# Autodesk Inventor assembly: STAGE1,ELEVATOR
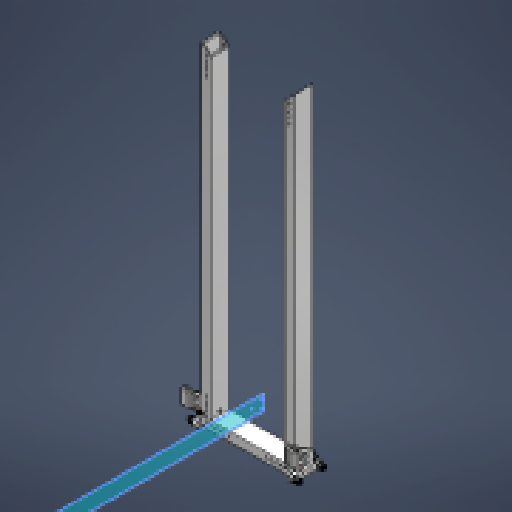
[picture p0: Inventor's stored thumbnail of the model, 512x512]
Saved by Autodesk Inventor 2024.3 (Build 283343000, 343)
## iProperties
ILogicPurgeVersion: 0.0.0.0
OnSaveVersion: 3.5.0.0
OnSaveAssembly: COREAutomationManager
Created: 2025-02-04
Part Number: STAGE1,ELEVATOR
Document SubType Name: Assembly
Designer: Jthib
Mfg Approved By: John.Thibert
Mass: 3994.13 g
Surface Area: 7109.04 cm^2
Volume: 1189.37 cm^3
Density: 3.3582 g/cm^3
ModelCat: Uncategorized
CN_MASS: 3.99
Author: Jthib
## Documents named in this file (12)
- \\clfs\homes\john.thibert\2025-Poseidon-Mechanical\STAGE1,ELEVATOR.iam
- \\clfs\homes\john.thibert\2025-Poseidon-Mechanical\TUBE,ELEVATOR,SIDE,STAGE1.ipt
- \\clfs\homes\john.thibert\2025-Poseidon-Mechanical\TUBE,ELEVATOR,BOT,STAGE1.ipt
- \\clfs\homes\john.thibert\2025-Poseidon-Mechanical\PLATE,BRACKET,ELEVATOR,STAGE1.ipt
- \\clfs\homes\john.thibert\2025-Poseidon-Mechanical\SLIDE,ELEVATOR,STAGE1,LH.iam
- \\clfs\homes\john.thibert\2025-Poseidon-Mechanical\SLIDE,ELEVATOR,STAGE1,RH.iam
- \\clfs\homes\john.thibert\2025-Poseidon-Mechanical\BRACE,CHAIN,#25,ELEVATOR.ipt
- \\clfs\homes\john.thibert\2025-Poseidon-Mechanical\BLOCK,BEARING,ARM,ELEVATOR.ipt
- \\clfs\homes\john.thibert\2025-Poseidon-Mechanical\60355K336_Ball Bearing.ipt
- \\clfs\homes\john.thibert\2025-Poseidon-Mechanical\91259A171_Alloy Steel Shoulder Screw.ipt
- \\clfs\homes\john.thibert\2025-Poseidon-Mechanical\BEARING,MOUNT,SIDE,ELEVATOR,MIRR.ipt
- \\clfs\homes\john.thibert\2025-Poseidon-Mechanical\BEARING,MOUNT,SIDE,ELEVATOR.ipt
## Components (19 placed, 13 different names)
1. SLIDE,ELEVATOR,STAGE1,LH.iam:1 [sub-assembly] — Mate:15, Mate:16, Mate:17, Mate:18
2. SLIDE,ELEVATOR,STAGE1,RH.iam:1 [sub-assembly]
3. TUBE,ELEVATOR,BOT,STAGE1.ipt:1 — Mate:14, Mate:19, Mate:20, Mate:22, Mate:23
4. TUBE,ELEVATOR,SIDE,STAGE1.ipt:1 — Mate:13, Mate:21, Mate:28, Mate:29, Mate:30
5. TUBE,ELEVATOR,SIDE,STAGE1.ipt:2 — Mate:24, Mate:25, Mate:26, Mate:27
6. BRACE,CHAIN,#25,ELEVATOR.ipt:1
7. PLATE,BRACKET,ELEVATOR,STAGE1.ipt:2
8. PLATE,BRACKET,ELEVATOR,STAGE1.ipt:1
9. BRACE,CHAIN,#25,ELEVATOR:2 — Mate:16, Mate:17, Mate:18
10. PLATE,BRACKET,ELEVATOR,STAGE1:4 — Mate:19, Mate:20, Mate:21
11. PLATE,BRACKET,ELEVATOR,STAGE1:5 — Mate:22, Mate:23, Mate:24
12. BLOCK,BEARING,ARM,ELEVATOR:1 — Mate:25, Mate:26, Mate:27
13. BEARING,MOUNT,SIDE,ELEVATOR:1
14. 91259A171_Alloy Steel Shoulder Screw:2
15. 60355K336_Ball Bearing:2
16. BEARING,MOUNT,SIDE,ELEVATOR,MIRR:1
17. 60355K336_Ball Bearing:1
18. 91259A171_Alloy Steel Shoulder Screw:1
19. BLOCK,BEARING,ARM,ELEVATOR:2 — Mate:28, Mate:29, Mate:30
## Relationships (47: Mate 37, Insert 10)
- [Insert]: TUBE,ELEVATOR,BOT,STAGE1.ipt:1 ↔ PLATE,BRACKET,ELEVATOR,STAGE1.ipt:1
- [Insert]: TUBE,ELEVATOR,BOT,STAGE1.ipt:1 ↔ PLATE,BRACKET,ELEVATOR,STAGE1.ipt:1
- [Insert]: TUBE,ELEVATOR,BOT,STAGE1.ipt:1 ↔ PLATE,BRACKET,ELEVATOR,STAGE1.ipt:2
- [Insert]: TUBE,ELEVATOR,BOT,STAGE1.ipt:1 ↔ PLATE,BRACKET,ELEVATOR,STAGE1.ipt:2
- [Insert]: TUBE,ELEVATOR,SIDE,STAGE1.ipt:2 ↔ PLATE,BRACKET,ELEVATOR,STAGE1.ipt:2
- [Insert]: TUBE,ELEVATOR,SIDE,STAGE1.ipt:2 ↔ PLATE,BRACKET,ELEVATOR,STAGE1.ipt:2
- [Insert]: TUBE,ELEVATOR,SIDE,STAGE1.ipt:1 ↔ PLATE,BRACKET,ELEVATOR,STAGE1.ipt:1
- [Insert]: TUBE,ELEVATOR,SIDE,STAGE1.ipt:1 ↔ PLATE,BRACKET,ELEVATOR,STAGE1.ipt:1
- [Mate]: SLIDE,ELEVATOR,STAGE1,RH.iam:1 ↔ TUBE,ELEVATOR,SIDE,STAGE1.ipt:2
- [Mate]: SLIDE,ELEVATOR,STAGE1,RH.iam:1 ↔ TUBE,ELEVATOR,SIDE,STAGE1.ipt:2
- [Mate]: SLIDE,ELEVATOR,STAGE1,RH.iam:1 ↔ TUBE,ELEVATOR,SIDE,STAGE1.ipt:2
- [Mate]: SLIDE,ELEVATOR,STAGE1,LH.iam:1 ↔ TUBE,ELEVATOR,SIDE,STAGE1.ipt:1
- [Mate]: SLIDE,ELEVATOR,STAGE1,LH.iam:1 ↔ TUBE,ELEVATOR,SIDE,STAGE1.ipt:1
- [Mate]: SLIDE,ELEVATOR,STAGE1,LH.iam:1 ↔ TUBE,ELEVATOR,SIDE,STAGE1.ipt:1
- [Mate]: SLIDE,ELEVATOR,STAGE1,RH.iam:1 ↔ BRACE,CHAIN,#25,ELEVATOR.ipt:1
- [Mate]: SLIDE,ELEVATOR,STAGE1,RH.iam:1 ↔ BRACE,CHAIN,#25,ELEVATOR.ipt:1
- [Mate]: SLIDE,ELEVATOR,STAGE1,RH.iam:1 ↔ BRACE,CHAIN,#25,ELEVATOR.ipt:1
- Mate:13 (-127 mm): TUBE,ELEVATOR,SIDE,STAGE1.ipt:1
- Mate:14 (-457.2 mm): TUBE,ELEVATOR,BOT,STAGE1.ipt:1
- Mate:15: SLIDE,ELEVATOR,STAGE1,LH.iam:1
- Mate:16: SLIDE,ELEVATOR,STAGE1,LH.iam:1 ↔ BRACE,CHAIN,#25,ELEVATOR:2
- Mate:17: SLIDE,ELEVATOR,STAGE1,LH.iam:1 ↔ BRACE,CHAIN,#25,ELEVATOR:2
- Mate:18: SLIDE,ELEVATOR,STAGE1,LH.iam:1 ↔ BRACE,CHAIN,#25,ELEVATOR:2
- Mate:19: TUBE,ELEVATOR,BOT,STAGE1.ipt:1 ↔ PLATE,BRACKET,ELEVATOR,STAGE1:4
- Mate:20: TUBE,ELEVATOR,BOT,STAGE1.ipt:1 ↔ PLATE,BRACKET,ELEVATOR,STAGE1:4
- Mate:21: TUBE,ELEVATOR,SIDE,STAGE1.ipt:1 ↔ PLATE,BRACKET,ELEVATOR,STAGE1:4
- Mate:22: TUBE,ELEVATOR,BOT,STAGE1.ipt:1 ↔ PLATE,BRACKET,ELEVATOR,STAGE1:5
- Mate:23: TUBE,ELEVATOR,BOT,STAGE1.ipt:1 ↔ PLATE,BRACKET,ELEVATOR,STAGE1:5
- Mate:24: TUBE,ELEVATOR,SIDE,STAGE1.ipt:2 ↔ PLATE,BRACKET,ELEVATOR,STAGE1:5
- Mate:25: TUBE,ELEVATOR,SIDE,STAGE1.ipt:2 ↔ BLOCK,BEARING,ARM,ELEVATOR:1
- Mate:26: TUBE,ELEVATOR,SIDE,STAGE1.ipt:2 ↔ BLOCK,BEARING,ARM,ELEVATOR:1
- Mate:27: TUBE,ELEVATOR,SIDE,STAGE1.ipt:2 ↔ BLOCK,BEARING,ARM,ELEVATOR:1
- Mate:28: TUBE,ELEVATOR,SIDE,STAGE1.ipt:1 ↔ BLOCK,BEARING,ARM,ELEVATOR:2
- Mate:29: TUBE,ELEVATOR,SIDE,STAGE1.ipt:1 ↔ BLOCK,BEARING,ARM,ELEVATOR:2
- Mate:30: TUBE,ELEVATOR,SIDE,STAGE1.ipt:1 ↔ BLOCK,BEARING,ARM,ELEVATOR:2
- [Mate]: 60355K336_Ball Bearing:1 ↔ 91259A171_Alloy Steel Shoulder Screw:1
- [Mate]: BRACE,CHAIN,#25,ELEVATOR.ipt:1 ↔ BEARING,MOUNT,SIDE,ELEVATOR,MIRR:1
- [Mate]: BRACE,CHAIN,#25,ELEVATOR.ipt:1 ↔ BEARING,MOUNT,SIDE,ELEVATOR,MIRR:1
- [Mate]: BRACE,CHAIN,#25,ELEVATOR.ipt:1 ↔ BEARING,MOUNT,SIDE,ELEVATOR,MIRR:1
- [Insert]: BEARING,MOUNT,SIDE,ELEVATOR,MIRR:1 ↔ 60355K336_Ball Bearing:1
- [Mate]: 60355K336_Ball Bearing:1 ↔ 91259A171_Alloy Steel Shoulder Screw:1
- [Mate]: 91259A171_Alloy Steel Shoulder Screw:2 ↔ 60355K336_Ball Bearing:2
- [Mate]: 91259A171_Alloy Steel Shoulder Screw:2 ↔ 60355K336_Ball Bearing:2
- [Insert]: BEARING,MOUNT,SIDE,ELEVATOR:1 ↔ 91259A171_Alloy Steel Shoulder Screw:2
- [Mate]: BRACE,CHAIN,#25,ELEVATOR:2 ↔ BEARING,MOUNT,SIDE,ELEVATOR:1
- [Mate]: BRACE,CHAIN,#25,ELEVATOR:2 ↔ BEARING,MOUNT,SIDE,ELEVATOR:1
- [Mate]: BRACE,CHAIN,#25,ELEVATOR:2 ↔ BEARING,MOUNT,SIDE,ELEVATOR:1
## Named parameters: d1097_d52 = 0 mm, d1156_d1097_d52 = 0 mm, d1158_d1102 = 0 mm
